# Autodesk Inventor assembly: copyingBrace
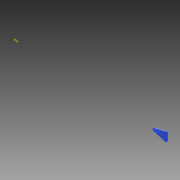
[picture p0: Inventor's stored thumbnail of the model, 180x180]
Saved by Autodesk Inventor 2013 (Build 170138000, 138)
## iProperties
Created: 2013-09-17
Part Number: copyingBrace
Document SubType Name: Assembly
Designer: Nano
Author: Nano
## Documents named in this file (3)
- C:\Users\Nano\Documents\InventorByron\InventorMasterProject\gyroPhone01\copyingBrace.iam
- C:\Users\Nano\Documents\InventorByron\InventorMasterProject\gyroPhone01\brace02.ipt
- C:\Users\Nano\Documents\InventorByron\InventorMasterProject\gyroPhone01\brace03.ipt
## Components (2 placed, 2 different names)
1. brace02:1 — Flush:1
2. brace03:1 — Flush:1
## Relationships (1: Flush 1)
- Flush:1: brace02:1 ↔ brace03:1
